# Autodesk Inventor assembly: FULL
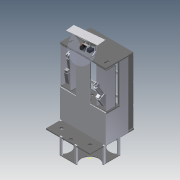
[picture p0: Inventor's stored thumbnail of the model, 180x180]
Saved by Autodesk Inventor 2011 (Build 150239000, 239)
## iProperties
Created: 2011-09-17
Part Number: FULL
Document SubType Name: Assembly
Designer: Matthew
Author: Matthew
## Documents named in this file (17)
- C:\Users\Matthew\Documents\matthew_autocad\prlite\FULL.iam
- C:\Users\Matthew\Documents\matthew_autocad\prlite\base\BASE.iam
- C:\Users\Matthew\Documents\matthew_autocad\prlite\inner torso\INNER TORSO.iam
- C:\Users\Matthew\Documents\matthew_autocad\prlite\slider\1.ipt
- C:\Users\Matthew\Documents\matthew_autocad\prlite\slider\2.ipt
- C:\Users\Matthew\Documents\matthew_autocad\prlite\outer torso\OUTER TORSO.iam
- C:\Users\Matthew\Documents\matthew_autocad\prlite\lazy susan\1.ipt
- C:\Users\Matthew\Documents\matthew_autocad\prlite\lazy susan\2.ipt
- C:\Users\Matthew\Documents\matthew_autocad\prlite\base\wheel connectors\small.ipt
- C:\Users\Matthew\Documents\matthew_autocad\prlite\base\wheel connectors\large.ipt
- C:\Users\Matthew\Documents\matthew_autocad\prlite\arm perhaps\linac body.ipt
- C:\Users\Matthew\Documents\matthew_autocad\prlite\arm perhaps\linac arm1.ipt
- C:\Users\Matthew\Documents\matthew_autocad\prlite\arm perhaps\linacconnect.ipt
- C:\Users\Matthew\Documents\matthew_autocad\prlite\base\wheel connectors\linac connector bar.ipt
- C:\Users\Matthew\Documents\matthew_autocad\prlite\base\wheel connectors\spacers.ipt
- C:\Users\Matthew\Documents\matthew_autocad\prlite\base\wheel connectors\linacspacers.ipt
- C:\Users\Matthew\Documents\matthew_autocad\prlite\head\HEAD.iam
## Components (32 placed, 20 different names)
1. BASE:1 [sub-assembly] — Mate:25, Mate:26, Mate:27, Mate:28, Mate:29, Mate:30, Mate:31, Mate:32, Mate:33, Mate:34, Mate:35, Mate:36, Mate:41, Flush:5, Mate:82, Mate:83, Flush:18, Flush:19, Mate:94, Flush:22, Flush:23
2. INNER TORSO:1 [sub-assembly] — Mate:8, Mate:15, Mate:16, Mate:40, Mate:41, Flush:5, Mate:56, Mate:59, Flush:23
3. slider1.1 — Mate:8, Mate:13, Mate:14, Flush:2, Mate:15, Mate:16, Mate:40, Flush:9
4. slider2.1 — Mate:13, Mate:14, Flush:2, Mate:37, Mate:38, Mate:39
5. 1:3 — Mate:23, Mate:24, Mate:66, Mate:67
6. 1:4 — Mate:21, Mate:22, Mate:73, Mate:74
7. 1:5 — Mate:19, Mate:20, Mate:71, Mate:72
8. 1:6 — Mate:17, Mate:18, Mate:64, Mate:65
9. 2:2 — Mate:17, Mate:18, Mate:30, Mate:31, Mate:32
10. 2:3 — Mate:21, Mate:22, Mate:28, Mate:33, Mate:34
11. 2:4 — Mate:19, Mate:20, Mate:29, Mate:35, Mate:36
12. 2:5 — Mate:23, Mate:24, Mate:25, Mate:26, Mate:27
13. OUTER TORSO:1 [sub-assembly] — Mate:37, Mate:38, Mate:39, Mate:60, Mate:61, Mate:62, Mate:63, Mate:100, Mate:101, Mate:102
14. slider1.2 — Mate:57, Mate:58, Flush:8, Mate:59, Flush:9, Flush:10
15. slider1.3 — Mate:54, Mate:55, Flush:7, Mate:56, Flush:10
16. slider2.2 — Mate:57, Mate:58, Flush:8, Mate:60, Mate:61
17. slider 2.3 — Mate:54, Mate:55, Flush:7, Mate:62, Mate:63
18. small:1 — Mate:66, Mate:67, Mate:69, Mate:70
19. small:2 — Mate:64, Mate:65, Mate:68
20. large:1 — Mate:68, Mate:69, Mate:70, Mate:75, Mate:76, Mate:84, Flush:19, Mate:86, Mate:87, Mate:88, Mate:91, Mate:92
21. small:3 — Mate:71, Mate:72, Mate:76, Mate:93
22. small:4 — Mate:73, Mate:74, Mate:75, Mate:89, Mate:90
23. linac body:1 — Mate:77, Mate:78, Mate:79, Flush:15
24. linac arm1:1 — Mate:79, Flush:15, Mate:80, Mate:81
25. linacconnect:1 — Mate:80, Mate:81, Mate:84, Mate:85, Flush:21, Mate:99
26. linacconnect:2 — Mate:77, Mate:78, Mate:82, Mate:83, Flush:18, Mate:95, Mate:96, Mate:97
27. linac connector bar:1 — Mate:85, Mate:86, Mate:87, Flush:21, Mate:99
28. spacers:1 — Mate:88, Mate:89, Mate:90
29. spacers:2 — Mate:91, Mate:92, Mate:93
30. linacspacers:1 — Mate:94, Flush:22, Mate:95, Mate:98
31. linacspacers:2 — Mate:96, Mate:97, Mate:98
32. HEAD:1 [sub-assembly] — Mate:100, Mate:101, Mate:102
## Relationships (91: Mate 79, Flush 12)
- Mate:8: INNER TORSO:1 ↔ slider1.1
- Mate:13: slider1.1 ↔ slider2.1
- Mate:14: slider1.1 ↔ slider2.1
- Flush:2: slider1.1 ↔ slider2.1
- Mate:15: INNER TORSO:1 ↔ slider1.1
- Mate:16: INNER TORSO:1 ↔ slider1.1
- Mate:17: 1:6 ↔ 2:2
- Mate:18: 1:6 ↔ 2:2
- Mate:19: 1:5 ↔ 2:4
- Mate:20: 1:5 ↔ 2:4
- Mate:21: 1:4 ↔ 2:3
- Mate:22: 1:4 ↔ 2:3
- Mate:23: 1:3 ↔ 2:5
- Mate:24: 1:3 ↔ 2:5
- Mate:25: BASE:1 ↔ 2:5
- Mate:26: BASE:1 ↔ 2:5
- Mate:27: BASE:1 ↔ 2:5
- Mate:28: BASE:1 ↔ 2:3
- Mate:29: BASE:1 ↔ 2:4
- Mate:30: BASE:1 ↔ 2:2
- Mate:31: BASE:1 ↔ 2:2
- Mate:32: BASE:1 ↔ 2:2
- Mate:33: BASE:1 ↔ 2:3
- Mate:34: BASE:1 ↔ 2:3
- Mate:35: BASE:1 ↔ 2:4
- Mate:36: BASE:1 ↔ 2:4
- Mate:37: slider2.1 ↔ OUTER TORSO:1
- Mate:38: slider2.1 ↔ OUTER TORSO:1
- Mate:39: slider2.1 ↔ OUTER TORSO:1
- Mate:40: INNER TORSO:1 ↔ slider1.1
- Mate:41: BASE:1 ↔ INNER TORSO:1
- Flush:5 (6.35 mm): BASE:1 ↔ INNER TORSO:1
- Mate:54: slider1.3 ↔ slider 2.3
- Mate:55: slider1.3 ↔ slider 2.3
- Flush:7: slider1.3 ↔ slider 2.3
- Mate:56: INNER TORSO:1 ↔ slider1.3
- Mate:57: slider1.2 ↔ slider2.2
- Mate:58: slider1.2 ↔ slider2.2
- Flush:8: slider1.2 ↔ slider2.2
- Mate:59: INNER TORSO:1 ↔ slider1.2
- Mate:60: OUTER TORSO:1 ↔ slider2.2
- Mate:61: OUTER TORSO:1 ↔ slider2.2
- Flush:9: slider1.1 ↔ slider1.2
- Mate:62: OUTER TORSO:1 ↔ slider 2.3
- Mate:63: OUTER TORSO:1 ↔ slider 2.3
- Flush:10: slider1.2 ↔ slider1.3
- Mate:64: 1:6 ↔ small:2
- Mate:65: 1:6 ↔ small:2
- Mate:66: 1:3 ↔ small:1
- Mate:67: 1:3 ↔ small:1
- Mate:68: small:2 ↔ large:1
- Mate:69 (8.4836 mm): small:1 ↔ large:1
- Mate:70: small:1 ↔ large:1
- Mate:71: 1:5 ↔ small:3
- Mate:72: 1:5 ↔ small:3
- Mate:73: 1:4 ↔ small:4
- Mate:74: 1:4 ↔ small:4
- Mate:75: large:1 ↔ small:4
- Mate:76: large:1 ↔ small:3
- Mate:77: linac body:1 ↔ linacconnect:2
- Mate:78 (1.11 mm): linac body:1 ↔ linacconnect:2
- Mate:79: linac body:1 ↔ linac arm1:1
- Flush:15: linac body:1 ↔ linac arm1:1
- Mate:80: linac arm1:1 ↔ linacconnect:1
- Mate:81 (3.65 mm): linac arm1:1 ↔ linacconnect:1
- Mate:82 (25.4 mm): BASE:1 ↔ linacconnect:2
- Mate:83 (-254 mm): BASE:1 ↔ linacconnect:2
- Mate:84 (3.175 mm): large:1 ↔ linacconnect:1
- Flush:18: BASE:1 ↔ linacconnect:2
- Flush:19 (199.644 mm): BASE:1 ↔ large:1
- Mate:85: linacconnect:1 ↔ linac connector bar:1
- Mate:86: large:1 ↔ linac connector bar:1
- Mate:87: large:1 ↔ linac connector bar:1
- Flush:21: linacconnect:1 ↔ linac connector bar:1
- Mate:88: large:1 ↔ spacers:1
- Mate:89: small:4 ↔ spacers:1
- Mate:90: small:4 ↔ spacers:1
- Mate:91: large:1 ↔ spacers:2
- Mate:92: large:1 ↔ spacers:2
- Mate:93: small:3 ↔ spacers:2
- Mate:94: BASE:1 ↔ linacspacers:1
- Flush:22: BASE:1 ↔ linacspacers:1
- Mate:95: linacconnect:2 ↔ linacspacers:1
- Mate:96: linacconnect:2 ↔ linacspacers:2
- Mate:97: linacconnect:2 ↔ linacspacers:2
- Mate:98: linacspacers:1 ↔ linacspacers:2
- Mate:99: linacconnect:1 ↔ linac connector bar:1
- Flush:23: BASE:1 ↔ INNER TORSO:1
- Mate:100: OUTER TORSO:1 ↔ HEAD:1
- Mate:101: OUTER TORSO:1 ↔ HEAD:1
- Mate:102: OUTER TORSO:1 ↔ HEAD:1
